# Autodesk Inventor assembly: UltraSonic Assembly
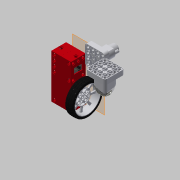
[picture p0: Inventor's stored thumbnail of the model, 180x180]
Saved by Autodesk Inventor 2019.3 (Build 233278000, 278)
## iProperties
Created: 2019-01-24
Part Number: UltraSonic Assembly
Document SubType Name: Assembly
Designer: Varga Daniel
Author: Varga Daniel
## Documents named in this file (5)
- C:\!_Dani\!_cloud\OneDrive\!_munka\Revolution\RevvyDemoKit\Structural parts\Demo parts\Caster wheel\Inventor imported\caster wheel design assy.iam
- C:\!_Dani\!_cloud\OneDrive\!_munka\Revolution\RevvyDemoKit\Structural parts\Demo parts\Wheel\Inventor imported\wheel_tyre.iam
- C:\!_Dani\!_cloud\OneDrive\!_munka\Revolution\RevvyDemoKit\Structural parts\Demo parts\Motor\Inventor imported\motor.iam
- C:\!_Dani\!_cloud\OneDrive\!_munka\Revolution\RevvyDemoKit\Structural parts\Demo parts\Caster wheel\Inventor imported\caster_wheel_1.iam
- C:\!_Dani\!_cloud\OneDrive\!_munka\Revolution\RevvyDemoKit\Structural parts\Demo parts\Caster wheel\Inventor imported\caster_wheel_2.iam
## Components (4 placed, 4 different names)
1. wheel_tyre:1 [sub-assembly] — Mate:136, Mate:137, Tangent:2
2. motor:1 [sub-assembly] — Mate:135, Mate:136, Mate:137, Angle:2
3. caster_wheel_2:1 [sub-assembly] — Flush:1
4. caster_wheel_1:1 [sub-assembly]
## Relationships (6: Mate 3, Angle 1, Tangent 1, Flush 1)
- Mate:135: motor:1
- Mate:136: wheel_tyre:1 ↔ motor:1
- Mate:137: wheel_tyre:1 ↔ motor:1
- Angle:2 (0 deg): motor:1
- Tangent:2: wheel_tyre:1
- Flush:1: caster_wheel_2:1
